# Autodesk Inventor assembly: Electrical Board - front bottom
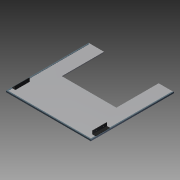
[picture p0: Inventor's stored thumbnail of the model, 180x180]
Saved by Autodesk Inventor 2012 (Build 160160000, 160)
## iProperties
Created: 2012-01-14
Part Number: Electrical Board - front bottom
Document SubType Name: Assembly
Designer: Antonella Wilby
Author: Antonella Wilby
## Documents named in this file (5)
- C:\Users\Antonella\Documents\GCC Robotics 2012 - Mechanical\Robot 2.0\Electrical\Front Electrical Board\Bottom\Electrical Board - front bottom.iam
- C:\Users\Antonella\Documents\GCC Robotics 2012 - Mechanical\Robot 2.0\Electrical\Front Electrical Board\Bottom\Electrical Board - front bottom.ipt
- C:\Users\Antonella\Documents\GCC Robotics 2012 - Mechanical\Robot 2.0\Electrical\Front Electrical Board\Bottom\front frame.ipt
- C:\Users\Antonella\Documents\GCC Robotics 2012 - Mechanical\Robot 2.0\Electrical\Front Electrical Board\Bottom\side frame.ipt
- C:\Users\Antonella\Documents\GCC Robotics 2012 - Mechanical\Robot 2.0\Electrical\Front Electrical Board\top board mount bracket.ipt
## Components (6 placed, 4 different names)
1. Electrical Board - front bottom:1 — Mate:1, Mate:2, Mate:3, Mate:4, Flush:1, Mate:5, Mate:6, Mate:7, Mate:8, Mate:9, Mate:10
2. front frame:1 — Mate:1, Mate:2, Mate:3
3. side frame:1 — Mate:4, Flush:1, Mate:5, Mate:12
4. side frame:2 — Mate:6, Mate:7, Mate:8, Mate:13
5. top board mount bracket:1 — Mate:9, Mate:12, Mate:14
6. top board mount bracket:2 — Mate:10, Mate:13, Mate:14
## Relationships (14: Mate 13, Flush 1)
- Mate:1: Electrical Board - front bottom:1 ↔ front frame:1
- Mate:2: Electrical Board - front bottom:1 ↔ front frame:1
- Mate:3: Electrical Board - front bottom:1 ↔ front frame:1
- Mate:4: Electrical Board - front bottom:1 ↔ side frame:1
- Flush:1: Electrical Board - front bottom:1 ↔ side frame:1
- Mate:5: Electrical Board - front bottom:1 ↔ side frame:1
- Mate:6: Electrical Board - front bottom:1 ↔ side frame:2
- Mate:7: Electrical Board - front bottom:1 ↔ side frame:2
- Mate:8: Electrical Board - front bottom:1 ↔ side frame:2
- Mate:9: Electrical Board - front bottom:1 ↔ top board mount bracket:1
- Mate:10: Electrical Board - front bottom:1 ↔ top board mount bracket:2
- Mate:12 (-28.575 mm): side frame:1 ↔ top board mount bracket:1
- Mate:13 (-28.575 mm): side frame:2 ↔ top board mount bracket:2
- Mate:14: top board mount bracket:1 ↔ top board mount bracket:2
